# Autodesk Inventor assembly: V0.2R1 Tulip Mod master v35
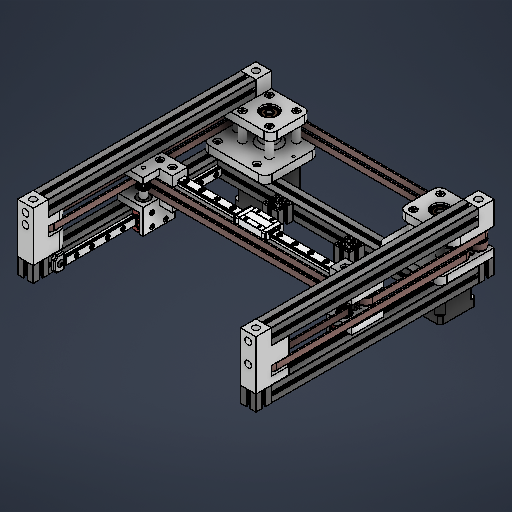
[picture p0: Inventor's stored thumbnail of the model, 512x512]
Saved by Autodesk Inventor 2026.1 (Build 301233020, 233B)
## iProperties
Created: 2025-05-23
Part Number: V0.2R1 Tulip Mod master v35
Document SubType Name: Assembly
Designer: Joshua Eah
Sending System: Autodesk Translation Framework v13.20.0.188
Preprocessor: ST-DEVELOPER v20
Title: V0.2R1 Tulip Mod master v35.step
## Documents named in this file (12)
- C:\Users\JoshuaEah\Documents\GitHub\Voron-0\CAD\Tulip - Machined Parts\Tulip Mod Master\Master Assembly.iam
- C:\Users\JoshuaEah\Documents\GitHub\Voron-0\CAD\Tulip - Machined Parts\Tulip Mod Master\Frame.iam
- C:\Users\JoshuaEah\Documents\GitHub\Voron-0\CAD\Tulip - Machined Parts\AB Drives\A Drive\A_Drive.iam
- C:\Users\JoshuaEah\Documents\GitHub\Voron-0\CAD\Tulip - Machined Parts\AB Drives\B Drive\B_Drive.iam
- C:\Users\JoshuaEah\Documents\GitHub\Voron-0\CAD\Tulip - Machined Parts\Tulip Mod Master\MGN7 Rail 150mm (1).iam
- C:\Users\JoshuaEah\Documents\GitHub\Voron-0\CAD\Tulip - Machined Parts\Tulip Mod Master\MGN7 Rail 150mm (2).iam
- C:\Users\JoshuaEah\Documents\GitHub\Voron-0\CAD\Tulip - Machined Parts\Tulip Mod Master\MGN7H Carriage (1).ipt
- C:\Users\JoshuaEah\Documents\GitHub\Voron-0\CAD\Tulip - Machined Parts\Tulip Mod Master\MGN7H Carriage (2).ipt
- C:\Users\JoshuaEah\Documents\GitHub\Voron-0\CAD\Tulip - Machined Parts\Tulip Mod Master\Belts.iam
- C:\Users\JoshuaEah\Documents\GitHub\Voron-0\CAD\Tulip - Machined Parts\Tulip Mod Master\X Axis.iam
- C:\Users\JoshuaEah\Documents\GitHub\Voron-0\CAD\Tulip - Machined Parts\Idlers\A Idler (Tulip) Assembly.iam
- C:\Users\JoshuaEah\Documents\GitHub\Voron-0\CAD\Tulip - Machined Parts\Idlers\B Idler (Tulip) Assembly.iam
## Components (11 placed, 11 different names)
1. Frame:1 [sub-assembly] — Insert:1, Angle:1, Angle:2, Angle:3, Flush:1, Flush:2, Mate:2, Mate:3, Mate:4, Mate:5, Insert:7, Insert:8, Insert:9, Insert:10, Insert:11
2. X Axis:1 [sub-assembly] — Insert:5, Insert:6, Transitional:1
3. A_Drive:1 [sub-assembly] — Insert:7
4. B_Drive:1 [sub-assembly] — Insert:1, Angle:1
5. MGN7 Rail 150mm (1):1 [sub-assembly] — Cylindrical:4, Cylindrical:2, Angle:2, Flush:2, Mate:2, Mate:5
6. MGN7 Rail 150mm (2):1 [sub-assembly] — Cylindrical:1, Cylindrical:3, Angle:3, Flush:1, Mate:3, Mate:4
7. MGN7H Carriage (1):1 — Cylindrical:4, Cylindrical:2, Insert:5
8. MGN7H Carriage (2):1 — Cylindrical:1, Cylindrical:3, Insert:6
9. Belts:1 [sub-assembly] — Transitional:1
10. A Idler (Tulip) Assembly:1 [sub-assembly] — Insert:8, Insert:9
11. B Idler (Tulip) Assembly:1 [sub-assembly] — Insert:10, Insert:11
## Relationships (22: Insert 8, CylindricalJoint 4, Mate 4, Angle 3, Flush 2, Transitional 1)
- Insert:1: Frame:1 ↔ B_Drive:1
- Angle:1 (0 deg): Frame:1 ↔ B_Drive:1
- Cylindrical:1: MGN7 Rail 150mm (2):1 ↔ MGN7H Carriage (2):1
- Cylindrical:4: MGN7 Rail 150mm (1):1 ↔ MGN7H Carriage (1):1
- Cylindrical:2: MGN7 Rail 150mm (1):1 ↔ MGN7H Carriage (1):1
- Cylindrical:3: MGN7 Rail 150mm (2):1 ↔ MGN7H Carriage (2):1
- Insert:5: X Axis:1 ↔ MGN7H Carriage (1):1
- Angle:2 (0 deg): Frame:1 ↔ MGN7 Rail 150mm (1):1
- Angle:3 (0 deg): Frame:1 ↔ MGN7 Rail 150mm (2):1
- Flush:1 (4 mm): Frame:1 ↔ MGN7 Rail 150mm (2):1
- Flush:2 (4 mm): Frame:1 ↔ MGN7 Rail 150mm (1):1
- Mate:2: Frame:1 ↔ MGN7 Rail 150mm (1):1
- Mate:3: Frame:1 ↔ MGN7 Rail 150mm (2):1
- Mate:4: Frame:1 ↔ MGN7 Rail 150mm (2):1
- Mate:5: Frame:1 ↔ MGN7 Rail 150mm (1):1
- Insert:6: X Axis:1 ↔ MGN7H Carriage (2):1
- Transitional:1: X Axis:1 ↔ Belts:1
- Insert:7: Frame:1 ↔ A_Drive:1
- Insert:8: Frame:1 ↔ A Idler (Tulip) Assembly:1
- Insert:9: Frame:1 ↔ A Idler (Tulip) Assembly:1
- Insert:10: Frame:1 ↔ B Idler (Tulip) Assembly:1
- Insert:11: Frame:1 ↔ B Idler (Tulip) Assembly:1
